# Autodesk Inventor assembly: PS20029
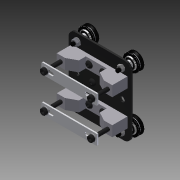
[picture p0: Inventor's stored thumbnail of the model, 180x180]
Saved by Autodesk Inventor 2014 (Build 180170000, 170)
## iProperties
Created: 2013-11-25
Part Number: PS20029
Document SubType Name: Assembly
Designer: Edward
Description: Spindle Carriage Assembly
Author: Edward
Title: Spindle Carriage Assembly
Subject: Shapeoko 2
## Documents named in this file (13)
- C:\Users\Edward\Documents\GitHub\Shapeoko_2\Autodesk_Inventor_Project\PS20029.iam
- C:\Users\Edward\Documents\GitHub\Shapeoko_2\Autodesk_Inventor_Project\30287-01.ipt
- C:\Users\Edward\Documents\GitHub\Shapeoko_2\Autodesk_Inventor_Project\PS20010.ipt
- C:\Users\Edward\Documents\GitHub\Shapeoko_2\Autodesk_Inventor_Project\25287-02.ipt
- C:\Users\Edward\Documents\GitHub\Shapeoko_2\Autodesk_Inventor_Project\25284-02.ipt
- C:\Users\Edward\Documents\GitHub\Shapeoko_2\Autodesk_Inventor_Project\PS20012.ipt
- C:\Users\Edward\Documents\GitHub\Shapeoko_2\Autodesk_Inventor_Project\30158-01.ipt
- C:\Users\Edward\Documents\GitHub\Shapeoko_2\Autodesk_Inventor_Project\25203-02.iam
- C:\Users\Edward\Documents\GitHub\Shapeoko_2\Autodesk_Inventor_Project\25312-14.ipt
- C:\Users\Edward\Documents\GitHub\Shapeoko_2\Autodesk_Inventor_Project\25286-05.ipt
- C:\Users\Edward\Documents\GitHub\Shapeoko_2\Autodesk_Inventor_Project\25286-02.ipt
- C:\Users\Edward\Documents\GitHub\Shapeoko_2\Autodesk_Inventor_Project\PS20013.ipt
- C:\Users\Edward\Documents\GitHub\Shapeoko_2\Autodesk_Inventor_Project\PS20005.ipt
## Components (46 placed, 12 different names)
1. 30287-01:1 — Insert:13, Insert:16, Insert:17, Insert:18, Insert:19
2. PS20010:1
3. PS20012:1 — Insert:14, Mate:5, Flush:3, Flush:4
4. 25286-02:1
5. 25286-02:6 — Insert:17
6. PS20012:2 — Insert:18, Insert:19, Mate:4, Flush:1, Flush:2, Mate:6
7. PS20013:1 — Mate:5, Flush:3, Flush:4
8. PS20013:2 — Mate:4, Flush:1, Flush:2, Mate:7
9. 25286-05:1
10. 30158-01:1
11. 25312-14:1
12. 25203-02:1 [sub-assembly]
13. 25286-05:2
14. 25203-02:2 [sub-assembly]
15. 25312-14:2 — Insert:13
16. 25284-02:1
17. 25287-02:1
18. 25286-05:3
19. 30158-01:2
20. 25312-14:3
21. 25203-02:3 [sub-assembly]
22. 25286-05:4
23. 25203-02:4 [sub-assembly]
24. 25312-14:4
25. 25284-02:2
26. 25287-02:2
27. 25284-02:3
28. 25287-02:3 — Insert:16
29. 25286-02:2 — Insert:14
30. 25284-02:4
31. 25287-02:4
32. 25286-02:3
33. 25284-02:5
34. 25287-02:5
35. 25286-02:4
36. 25284-02:6
37. 25287-02:6
38. 25286-02:5
39. PS20005:1 — Mate:6
40. 25287-02:7 — Mate:7
41. PS20005:2
42. 25287-02:8
43. PS20005:3
44. 25287-02:9
45. PS20005:4
46. 25287-02:10
## Component patterns: (2 elements, first: 25286-05:1 + 30158-01:1 + 25312-14:1 + 25203-02:1 + 25286-05:2 + 25203-02:2 + 25312-14:2 + 25284-02:1 + 25287-02:1), (4 elements, first: 25284-02:3 + 25287-02:3 + 25286-02:2), (4 elements, first: PS20005:1 + 25287-02:7)
## Relationships (31: Insert 20, Mate 7, Flush 4)
- [Insert]: 30287-01:1 ↔ PS20010:1
- [Insert]: 30287-01:1 ↔ PS20010:1
- [Insert]: 30287-01:1 ↔ 25287-02:1
- [Insert]: 25284-02:1 ↔ 25287-02:1
- [Insert]: 30287-01:1 ↔ PS20012:1
- [Insert]: 30287-01:1 ↔ PS20012:1
- [Insert]: 25312-14:1 ↔ 25203-02:1
- [Insert]: 25286-05:1 ↔ 25203-02:1
- [Mate]: 30158-01:1 ↔ 25312-14:1
- [Insert]: 30287-01:1 ↔ 30158-01:1
- [Mate]: 30158-01:1 ↔ 25312-14:1
- [Mate]: 30287-01:1 ↔ 25312-14:1
- [Insert]: 30287-01:1 ↔ 25286-02:1
- [Insert]: 25203-02:2 ↔ 25312-14:2
- [Insert]: 25286-05:2 ↔ 25203-02:2
- Insert:13: 30287-01:1 ↔ 25312-14:2
- Insert:14: PS20012:1 ↔ 25286-02:2
- [Insert]: 25284-02:3 ↔ 25287-02:3
- Insert:16: 30287-01:1 ↔ 25287-02:3
- Insert:17: 30287-01:1 ↔ 25286-02:6
- Insert:18: 30287-01:1 ↔ PS20012:2
- Insert:19: 30287-01:1 ↔ PS20012:2
- [Insert]: PS20005:1 ↔ 25287-02:7
- Mate:4 (20 mm): PS20012:2 ↔ PS20013:2
- Flush:1: PS20012:2 ↔ PS20013:2
- Flush:2: PS20012:2 ↔ PS20013:2
- Mate:5 (20 mm): PS20012:1 ↔ PS20013:1
- Flush:3: PS20012:1 ↔ PS20013:1
- Flush:4: PS20012:1 ↔ PS20013:1
- Mate:6: PS20012:2 ↔ PS20005:1
- Mate:7: PS20013:2 ↔ 25287-02:7
## Named parameters: d267_d259_d246 = 0 mm, d268_d260_d247 = 0 mm, d269_d262 = 0 mm, d13_d267_d259_d246 = 0 mm, d14_d268_d260_d247 = 0 mm, d21_d249 = 0 mm, d331_d137 = 0 mm
